# Autodesk Inventor assembly: ASM PI Print Server
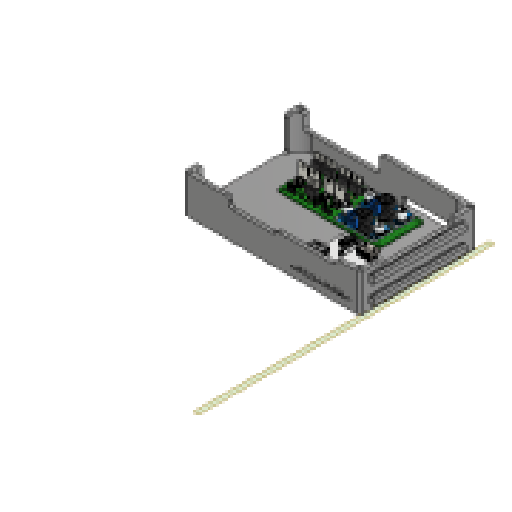
[picture p0: Inventor's stored thumbnail of the model, 512x512]
Saved by Autodesk Inventor 2023 (Build 270158000, 158)
## iProperties
Created: 2023-03-16
Part Number: ASM PI Print Server
Document SubType Name: Assembly
Designer: alber
Author: alber
## Documents named in this file (3)
- C:\Users\alber\Desktop\Files\Ender3-Upgrade\CAD\ASM PI Print Server.iam
- C:\Users\alber\Desktop\Files\Ender3-Upgrade\CAD\RaspberryPi 3 A+.iam
- C:\Users\alber\Desktop\Files\Ender3-Upgrade\CAD\Back_Case.ipt
## Components (2 placed, 2 different names)
1. Back_Case:1
2. RaspberryPi 3 A+:1 [sub-assembly]
## Relationships (2: Mate 1, Angle 1)
- [Mate] (5 mm): Back_Case:1 ↔ RaspberryPi 3 A+:1
- [Angle] (0 deg): Back_Case:1 ↔ RaspberryPi 3 A+:1
